# Autodesk Inventor assembly: steering_stand
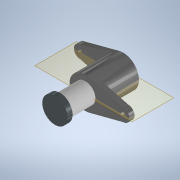
[picture p0: Inventor's stored thumbnail of the model, 180x180]
Saved by Autodesk Inventor 2020 (Build 240168000, 168)
## iProperties
Created: 2020-03-09
Part Number: steering_stand
Document SubType Name: Assembly
Designer: 0x6f736f646f
Author: 0x6f736f646f
## Documents named in this file (4)
- C:\Users\0x6f736f646f\Documents\Inventor\Eureka_Autonomous_CAR\steering_stand.iam
- C:\Users\0x6f736f646f\Documents\Inventor\Eureka_Autonomous_CAR\steering_stand_off.ipt
- C:\Users\0x6f736f646f\Documents\Inventor\Eureka_Autonomous_CAR\steering_stand_off_bush.ipt
- C:\Users\0x6f736f646f\Documents\Inventor\Eureka_Autonomous_CAR\steering_stand_off_pin.ipt
## Components (3 placed, 3 different names)
1. steering_stand_off:1 — Mate:3, Mate:4, Mate:5
2. steering_stand_off_bush:1 — Mate:1, Mate:2, Mate:3, Mate:4, Mate:5
3. steering_stand_off_pin:1 — Mate:1, Mate:2
## Relationships (5: Mate 5)
- Mate:1: steering_stand_off_bush:1 ↔ steering_stand_off_pin:1
- Mate:2: steering_stand_off_bush:1 ↔ steering_stand_off_pin:1
- Mate:3: steering_stand_off:1 ↔ steering_stand_off_bush:1
- Mate:4: steering_stand_off:1 ↔ steering_stand_off_bush:1
- Mate:5: steering_stand_off:1 ↔ steering_stand_off_bush:1
